# Autodesk Inventor assembly: ChassisDes1
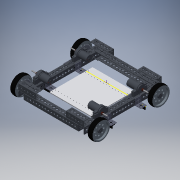
[picture p0: Inventor's stored thumbnail of the model, 180x180]
Saved by Autodesk Inventor 2016 (Build 200138000, 138)
## iProperties
Created: 2015-08-30
Part Number: ChassisDes1
Document SubType Name: Assembly
Designer: Tim
Author: Tim
## Documents named in this file (9)
- C:\Users\Tim\Documents\GitHub\phi_robotics\3d-models\FTC_Tetrix_KOP_Block_Party\Tim Bloot Designs\ChassisDes1.iam
- C:\Users\Tim\Documents\GitHub\phi_robotics\3d-models\FTC_Tetrix_KOP_Block_Party\Tim Bloot Designs\RollingSquareC1.iam
- C:\Users\Tim\Documents\GitHub\phi_robotics\3d-models\FTC_Tetrix_KOP_Block_Party\Tetrix_Kit_FTC\Autodesk Inventor Files\tetrix_corner_bracket.ipt
- C:\Users\Tim\Documents\GitHub\phi_robotics\3d-models\FTC_Tetrix_KOP_Block_Party\Tim Bloot Designs\customLbeam.ipt
- C:\Users\Tim\Documents\GitHub\phi_robotics\3d-models\FTC_Tetrix_KOP_Block_Party\Tetrix_Kit_FTC\Autodesk Inventor Files\tetrix_c_channel-4.ipt
- C:\Users\Tim\Documents\GitHub\phi_robotics\3d-models\FTC_Tetrix_KOP_Block_Party\Tetrix_Kit_FTC\Autodesk Inventor Files\tetrix_c_channel-2.ipt
- C:\Users\Tim\Documents\GitHub\phi_robotics\3d-models\FTC_Tetrix_KOP_Block_Party\Tim Bloot Designs\CustomBasePlate.ipt
- C:\Users\Tim\Documents\GitHub\phi_robotics\3d-models\FTC_Tetrix_KOP_Block_Party\Tetrix_Kit_FTC\Autodesk Inventor Files\tetrix_motor_mount-old.ipt
- C:\Users\Tim\Documents\GitHub\phi_robotics\3d-models\FTC_Tetrix_KOP_Block_Party\Tetrix_Kit_FTC\Autodesk Inventor Files\tetrix_motor.iam
## Components (27 placed, 8 different names)
1. tetrix_corner_bracket:1 — Rigid:2, Rigid:33
2. tetrix_corner_bracket:2 — Rigid:1
3. RollingSquareC1:1 [sub-assembly] — Rigid:1, Rigid:2, Rigid:16, Rigid:17, Rigid:22, Rigid:25, Rigid:27, Rigid:28
4. RollingSquareC1:2 [sub-assembly] — Rigid:9, Rigid:10, Rigid:18, Rigid:19, Rigid:23, Rigid:26, Rigid:29, Rotational:32
5. tetrix_corner_bracket:7 — Rigid:9, Rigid:32
6. tetrix_corner_bracket:8 — Rigid:10
7. customLbeam:3 — Rigid:32, Rigid:33
8. customLbeam:4 — Rigid:30, Rigid:31
9. tetrix_corner_bracket:9 — Rigid:16
10. tetrix_corner_bracket:10 — Rigid:17, Rigid:31
11. tetrix_corner_bracket:11 — Rigid:19, Rigid:30
12. tetrix_corner_bracket:12 — Rigid:18
13. tetrix_c_channel-4:1 — Rigid:24
14. tetrix_c_channel-4:2 — Rotational:28
15. tetrix_c_channel-2:1 — Rigid:22, Rigid:24
16. tetrix_c_channel-2:2 — Rigid:23
17. tetrix_c_channel-2:3 — Rigid:25
18. tetrix_c_channel-2:4 — Rigid:26, Rotational:28
19. CustomBasePlate:1
20. tetrix_motor_mount-old:1 — Rigid:27, Rotational:29
21. tetrix_motor:1 [sub-assembly] — Rotational:29
22. tetrix_motor_mount-old:2 — Rigid:28, Rotational:30
23. tetrix_motor:2 [sub-assembly] — Rotational:30
24. tetrix_motor_mount-old:3 — Rigid:29, Rotational:31
25. tetrix_motor:3 [sub-assembly] — Rotational:31
26. tetrix_motor_mount-old:4 — Rotational:32, Rotational:33
27. tetrix_motor:4 [sub-assembly] — Rotational:33
## Relationships (26: WeldJoint 20, RevoluteJoint 6)
- Rigid:1 [WeldJoint]: tetrix_corner_bracket:2 ↔ RollingSquareC1:1
- Rigid:2 [WeldJoint]: tetrix_corner_bracket:1 ↔ RollingSquareC1:1
- Rigid:9 [WeldJoint]: RollingSquareC1:2 ↔ tetrix_corner_bracket:7
- Rigid:10 [WeldJoint]: RollingSquareC1:2 ↔ tetrix_corner_bracket:8
- Rigid:16 [WeldJoint]: RollingSquareC1:1 ↔ tetrix_corner_bracket:9
- Rigid:17 [WeldJoint]: RollingSquareC1:1 ↔ tetrix_corner_bracket:10
- Rigid:18 [WeldJoint]: RollingSquareC1:2 ↔ tetrix_corner_bracket:12
- Rigid:19 [WeldJoint]: RollingSquareC1:2 ↔ tetrix_corner_bracket:11
- Rigid:22 [WeldJoint]: RollingSquareC1:1 ↔ tetrix_c_channel-2:1
- Rigid:23 [WeldJoint]: RollingSquareC1:2 ↔ tetrix_c_channel-2:2
- Rigid:24 [WeldJoint]: tetrix_c_channel-4:1 ↔ tetrix_c_channel-2:1
- Rigid:25 [WeldJoint]: RollingSquareC1:1 ↔ tetrix_c_channel-2:3
- Rigid:26 [WeldJoint]: RollingSquareC1:2 ↔ tetrix_c_channel-2:4
- Rotational:28 [RevoluteJoint]: tetrix_c_channel-4:2 ↔ tetrix_c_channel-2:4
- Rigid:27 [WeldJoint]: RollingSquareC1:1 ↔ tetrix_motor_mount-old:1
- Rotational:29 [RevoluteJoint]: tetrix_motor_mount-old:1 ↔ tetrix_motor:1
- Rigid:28 [WeldJoint]: RollingSquareC1:1 ↔ tetrix_motor_mount-old:2
- Rotational:30 [RevoluteJoint]: tetrix_motor_mount-old:2 ↔ tetrix_motor:2
- Rigid:29 [WeldJoint]: RollingSquareC1:2 ↔ tetrix_motor_mount-old:3
- Rotational:31 [RevoluteJoint]: tetrix_motor_mount-old:3 ↔ tetrix_motor:3
- Rotational:32 [RevoluteJoint]: RollingSquareC1:2 ↔ tetrix_motor_mount-old:4
- Rotational:33 [RevoluteJoint]: tetrix_motor_mount-old:4 ↔ tetrix_motor:4
- Rigid:30 [WeldJoint]: customLbeam:4 ↔ tetrix_corner_bracket:11
- Rigid:31 [WeldJoint]: customLbeam:4 ↔ tetrix_corner_bracket:10
- Rigid:32 [WeldJoint]: tetrix_corner_bracket:7 ↔ customLbeam:3
- Rigid:33 [WeldJoint]: tetrix_corner_bracket:1 ↔ customLbeam:3
## Named parameters: d9_d4 = 0 mm, d10_d8 = 0 mm
